# Autodesk Inventor assembly: 2016-02-19-RobotV20iam
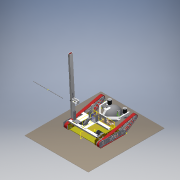
[picture p0: Inventor's stored thumbnail of the model, 180x180]
Saved by Autodesk Inventor 2017 (Build 210142000, 142)
## iProperties
Created: 2016-02-10
Part Number: 2016-02-19-RobotV20iam
Document SubType Name: Assembly
Designer: steele
Author: steele
## Documents named in this file (21)
- C:\snobotics\CAD-Development\robSteele\SnoBotics2016\2016-02-19-RobotV20\2016-02-19-RobotV20iam.iam
- C:\snobotics\CAD-Development\robSteele\SnoBotics2016\RhinoTrackDriveModule\am-3322+RhinoTrackDriveModule.iam
- C:\snobotics\CAD-Development\robSteele\SnoBotics2016\RhinoBottomFloorOptions\SheetBottomFloorV01.ipt
- C:\snobotics\CAD-Development\robSteele\SnoBotics2016\RhinoBottomFloorOptions\Floor.ipt
- C:\snobotics\CAD-Development\robSteele\SnoBotics2016\DraftOfBoulder.ipt
- C:\snobotics\CAD-Development\robSteele\SnoBotics2016\2016-05-05-ShooterPrototype\SupportPlateMotorMountV01.ipt
- C:\snobotics\CAD-Development\robSteele\SnoBotics2016\2016-05-05-ShooterPrototype\SupportPlateWithPostOnlyV01.ipt
- C:\snobotics\CAD-Development\robSteele\SnoBotics2016\2016-05-05-ShooterPrototype\SnowBlowerMotorMountAndHub.iam
- C:\snobotics\CAD-Development\robSteele\SnoBotics2016\2016-05-05-ShooterPrototype\ShooterAssemblyForRobotV16.iam
- C:\snobotics\CAD-Development\robSteele\SnoBotics2016\AM Parts\SnowBlowerMotorAndMount.iam
- C:\snobotics\CAD-Development\robSteele\SnoBotics2016\2016-02-12-RhinoSheetMetalStartOfLift\2016-02-12-RobotV17\Design Accelerator\Chain Drive1.iam
- C:\snobotics\CAD-Development\robSteele\SnoBotics2016\2016-01-31-Lift\BasePostForSideOfRobot.ipt
- C:\snobotics\CAD-Development\robSteele\SnoBotics2016\2016-01-31-Lift\rearAxel.ipt
- C:\snobotics\CAD-Development\robSteele\SnoBotics2016\2016-02-12-RhinoSheetMetalStartOfLift\2016-02-12-RobotV17\Design Accelerator\Chain Drive2.iam
- C:\snobotics\CAD-Development\robSteele\SnoBotics2016\2016-01-31-Lift\MiddlePostsForTwoSprockets.ipt
- C:\snobotics\CAD-Development\robSteele\SnoBotics2016\RhinoTrackDriveModule\am-3322+RhinoTrackDriveModule_MIR15.iam
- C:\snobotics\CAD-Development\robSteele\SnoBotics2016\TelescopeArm\TelescopingArm.iam
- C:\snobotics\CAD-Development\robSteele\SnoBotics2016\RobotVolume\RhinoV19MaxVolume.ipt
- C:\snobotics\CAD-Development\robSteele\SnoBotics2016\2016-02-19-RobotV20\1556A540.ipt
- C:\snobotics\CAD-Development\robSteele\SnoBotics2016\2016-02-12-RhinoSheetMetalStartOfLift\1x2_alumTubing.ipt
- C:\snobotics\CAD-Development\robSteele\SnoBotics2016\2016-02-12-RhinoSheetMetalStartOfLift\sheetPlateForBase.ipt
## Components (23 placed, 19 different names)
1. am-3322+RhinoTrackDriveModule:1 [sub-assembly] — Mate:1, Flush:1, Flush:2, Mate:4, Insert:1, Insert:2
2. SheetBottomFloorV01:1 — Mate:1, Flush:1, Flush:2, Mate:2, Mate:3, Flush:6, Flush:8, Mate:28, Mate:33, Mate:49, Mate:53
3. Floor:1 — Mate:2, Mate:3, Mate:4, Flush:7, Mate:5, Mate:50
4. DraftOfBoulder:1 — Flush:6, Flush:7, Mate:5, Mate:34
5. SupportPlateMotorMountV01:1
6. SupportPlateWithPostOnlyV01:1
7. SnowBlowerMotorMountAndHub:1 [sub-assembly]
8. ShooterAssemblyForRobotV16:1 [sub-assembly] — Mate:33, Mate:34
9. SnowBlowerMotorAndMount:1 [sub-assembly]
10. Chain Drive:1 [sub-assembly]
11. BasePostForSideOfRobot:1 — Mate:56, Flush:16, Flush:17, Insert:3
12. rearAxel:1
13. Chain Drive:2 [sub-assembly]
14. MiddlePostsForTwoSprockets:1 — Mate:28
15. am-3322+RhinoTrackDriveModule_MIR15:1 [sub-assembly]
16. TelescopingArm:1 [sub-assembly] — Insert:3
17. RhinoV19MaxVolume:1 — Mate:49, Mate:50
18. 1556A540:1 — Insert:1, Mate:51, Flush:9, Flush:10
19. 1556A540:2 — Insert:2, Mate:52, Flush:11, Flush:12
20. 1x2_alumTubing:1 — Mate:51, Flush:9, Flush:10, Mate:54, Flush:13, Mate:55, Flush:14, Flush:15
21. 1x2_alumTubing:2 — Mate:52, Flush:11, Flush:12, Mate:57
22. sheetPlateForBase:1 — Mate:53, Mate:54, Flush:13
23. sheetPlateForBase:2 — Mate:55, Flush:14, Flush:15, Mate:56, Flush:16, Flush:17, Mate:57
## Relationships (34: Mate 17, Flush 14, Insert 3)
- Mate:1: am-3322+RhinoTrackDriveModule:1 ↔ SheetBottomFloorV01:1
- Flush:1: am-3322+RhinoTrackDriveModule:1 ↔ SheetBottomFloorV01:1
- Flush:2 (4.7625 mm): am-3322+RhinoTrackDriveModule:1 ↔ SheetBottomFloorV01:1
- Mate:2: SheetBottomFloorV01:1 ↔ Floor:1
- Mate:3: SheetBottomFloorV01:1 ↔ Floor:1
- Mate:4 (0.889 mm): am-3322+RhinoTrackDriveModule:1 ↔ Floor:1
- Flush:6: SheetBottomFloorV01:1 ↔ DraftOfBoulder:1
- Flush:7 (127 mm): Floor:1 ↔ DraftOfBoulder:1
- Mate:5 (-381 mm): Floor:1 ↔ DraftOfBoulder:1
- Flush:8: SheetBottomFloorV01:1
- Mate:28: SheetBottomFloorV01:1 ↔ MiddlePostsForTwoSprockets:1
- Mate:33: SheetBottomFloorV01:1 ↔ ShooterAssemblyForRobotV16:1
- Mate:34: DraftOfBoulder:1 ↔ ShooterAssemblyForRobotV16:1
- Mate:49: SheetBottomFloorV01:1 ↔ RhinoV19MaxVolume:1
- Mate:50: Floor:1 ↔ RhinoV19MaxVolume:1
- Insert:1: am-3322+RhinoTrackDriveModule:1 ↔ 1556A540:1
- Insert:2: am-3322+RhinoTrackDriveModule:1 ↔ 1556A540:2
- Mate:51: 1556A540:1 ↔ 1x2_alumTubing:1
- Flush:9: 1556A540:1 ↔ 1x2_alumTubing:1
- Flush:10: 1556A540:1 ↔ 1x2_alumTubing:1
- Mate:52: 1556A540:2 ↔ 1x2_alumTubing:2
- Flush:11: 1556A540:2 ↔ 1x2_alumTubing:2
- Flush:12: 1556A540:2 ↔ 1x2_alumTubing:2
- Mate:53: SheetBottomFloorV01:1 ↔ sheetPlateForBase:1
- Mate:54: 1x2_alumTubing:1 ↔ sheetPlateForBase:1
- Flush:13 (-25.4 mm): 1x2_alumTubing:1 ↔ sheetPlateForBase:1
- Mate:55: 1x2_alumTubing:1 ↔ sheetPlateForBase:2
- Flush:14 (50.8 mm): 1x2_alumTubing:1 ↔ sheetPlateForBase:2
- Flush:15 (-25.4 mm): 1x2_alumTubing:1 ↔ sheetPlateForBase:2
- Mate:56: BasePostForSideOfRobot:1 ↔ sheetPlateForBase:2
- Flush:16: BasePostForSideOfRobot:1 ↔ sheetPlateForBase:2
- Flush:17: BasePostForSideOfRobot:1 ↔ sheetPlateForBase:2
- Insert:3: BasePostForSideOfRobot:1 ↔ TelescopingArm:1
- Mate:57: 1x2_alumTubing:2 ↔ sheetPlateForBase:2
## Named parameters: OffsetBetweenFloorAndLeftTred = 0.889 mm
